# Autodesk Inventor assembly: IR-plate
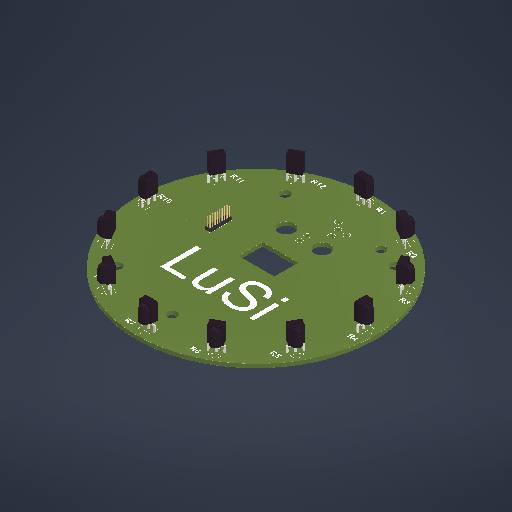
[picture p0: Inventor's stored thumbnail of the model, 512x512]
Saved by Autodesk Inventor 2026.1 (Build 301233000, 233)
## iProperties
Company: Kicad
Created: 2026-04-13
Part Number: IR-plate
Description: KiCad electronic assembly
Document SubType Name: Assembly
Designer: Familie
Authority: Unknown
Sending System: KiCad to STEP converter
Preprocessor: Open CASCADE STEP processor 7.9
Title: Roboter neu.step
Author: Pcbnew
## Documents named in this file (8)
- C:\Users\Familie\Documents\Luka\Robocup Soccer\Wien\final\IR-plate.iam
- C:\Users\Familie\Documents\Luka\KiCad\IR-Platte\Roboter neu\Roboter neu\Roboter neu\Vishay_MINICAST-3Pin.ipt
- C:\Users\Familie\Documents\Luka\KiCad\IR-Platte\Roboter neu\Roboter neu\Roboter neu\PinHeader_2x09_P1.00mm_Vertical.ipt
- C:\Users\Familie\Documents\Luka\KiCad\IR-Platte\Roboter neu\Roboter neu\Roboter neu\Roboter neu_silkscreen.ipt
- C:\Users\Familie\Documents\Luka\KiCad\IR-Platte\Roboter neu\Roboter neu\Roboter neu\Roboter neu_silkscreen_1.ipt
- C:\Users\Familie\Documents\Luka\KiCad\IR-Platte\Roboter neu\Roboter neu\Roboter neu\Roboter neu_soldermask.ipt
- C:\Users\Familie\Documents\Luka\KiCad\IR-Platte\Roboter neu\Roboter neu\Roboter neu\Roboter neu_soldermask_1.ipt
- C:\Users\Familie\Documents\Luka\KiCad\IR-Platte\Roboter neu\Roboter neu\Roboter neu\Roboter neu_PCB.ipt
## Components (18 placed, 18 different names)
1. 1
2. 2
3. 3
4. 4
5. 5
6. 6
7. 7
8. 8
9. 9
10. 10
11. 11
12. 12
13. 13
14. 14
15. 15
16. 16
17. 17
18. 18
## Named parameters: Finish1_Area = 155.6, Finish2_Area = 155.6, Finish3_Area = 2.63072, Finish4_Area = 2.62406
note: some values were not read from the file. Shown as the stored number, unit unknown: "Finish1_Area", "Finish2_Area", "Finish3_Area", "Finish4_Area".
